# Autodesk Inventor assembly: ZLAC8015D V4.0
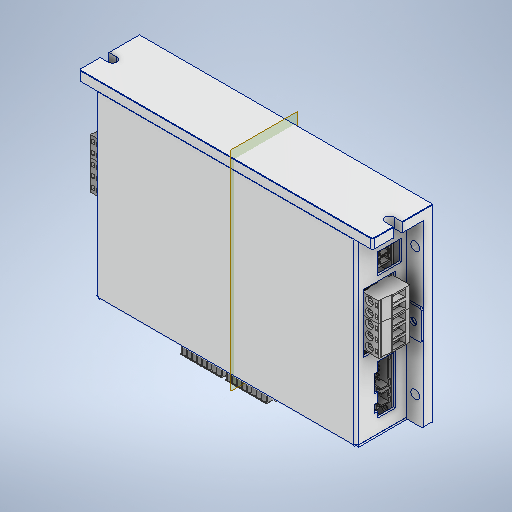
[picture p0: Inventor's stored thumbnail of the model, 512x512]
Saved by Autodesk Inventor 2026.2 (Build 302298010, 298A)
## iProperties
Created: 2025-03-11
Part Number: ZLAC8015D V4.0
Description: STEP AP203
Document SubType Name: Assembly
Designer: chanh
Sending System: SolidWorks 2020
Preprocessor: SwSTEP 2.0
Title: ZLAC8015D-V4_0-20250311.STEP
Revision Number: ÈÎºÎ
## Documents named in this file (5)
- C:\Users\chanh\내 드라이브\교과공부\2026년 1학기 (4학년 1학기)\01창의제품설계\CLOSE_hardware\00부품\ZLAC8015D V4.0 (드라이버)\ZLAC8015D V4.0.iam
- C:\Users\chanh\내 드라이브\교과공부\2026년 1학기 (4학년 1학기)\01창의제품설계\CLOSE_hardware\00부품\ZLAC8015D V4.0 (드라이버)\dizuo5.ipt
- C:\Users\chanh\내 드라이브\교과공부\2026년 1학기 (4학년 1학기)\01창의제품설계\CLOSE_hardware\00부품\ZLAC8015D V4.0 (드라이버)\tongzhu.ipt
- C:\Users\chanh\내 드라이브\교과공부\2026년 1학기 (4학년 1학기)\01창의제품설계\CLOSE_hardware\00부품\ZLAC8015D V4.0 (드라이버)\8015D7-PCB.iam
- C:\Users\chanh\내 드라이브\교과공부\2026년 1학기 (4학년 1학기)\01창의제품설계\CLOSE_hardware\00부품\ZLAC8015D V4.0 (드라이버)\8015D-G É°³ÈÉ« V4_0-20241206.ipt
## Components (9 placed, 9 different names)
1. dizuo5_1 — Symmetry:1
2. tongzhu_2
3. tongzhu_3
4. tongzhu_4
5. tongzhu_5
6. 8015D7-PCB_6 [sub-assembly]
7. tongzhu_7
8. tongzhu_8
9. 8015D-G É°³ÈÉ« V4_0-20241206_9 — Symmetry:1
## Relationships (1: Symmetry 1)
- Symmetry:1: dizuo5_1 ↔ 8015D-G É°³ÈÉ« V4_0-20241206_9
